# Autodesk Inventor assembly: Assembly2
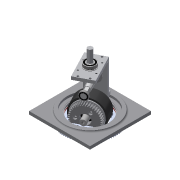
[picture p0: Inventor's stored thumbnail of the model, 180x180]
Saved by Autodesk Inventor 2014 SP1 (Build 180222100, 222)
## iProperties
Created: 2014-04-22
Part Number: Assembly2
Document SubType Name: Assembly
Designer: Rauhul Varma
Author: Rauhul Varma
## Documents named in this file (28)
- C:\Users\Rauhul Varma\Desktop\GRT 2013-2014 Designs\Low CoG Swerve\Assembly2.iam
- C:\Users\Rauhul Varma\Desktop\GRT 2013-2014 Designs\Low CoG Swerve\84T 20 DP Gear.ipt
- C:\Users\Rauhul Varma\Desktop\GRT 2013-2014 Designs\Low CoG Swerve\Module Side Beam.ipt
- C:\Users\Rauhul Varma\Desktop\GRT 2013-2014 Designs\Low CoG Swerve\Wheel.ipt
- C:\Users\Rauhul Varma\Desktop\GRT 2013-2014 Designs\Low CoG Swerve\6901-2RS.ipt
- C:\Users\Rauhul Varma\Desktop\GRT 2013-2014 Designs\Low CoG Swerve\Dead Axle.ipt
- C:\Users\Rauhul Varma\Desktop\GRT 2013-2014 Designs\Low CoG Swerve\FBHCS .25-20 .500 Length.ipt
- C:\Users\Rauhul Varma\Desktop\GRT 2013-2014 Designs\Low CoG Swerve\SHCS LP 8-32 .7500 Long.ipt
- C:\Users\Rauhul Varma\Desktop\GRT 2013-2014 Designs\Low CoG Swerve\SHCS 6-32 .5000 Long.ipt
- C:\Users\Rauhul Varma\Desktop\GRT 2013-2014 Designs\Low CoG Swerve\Dead Axle Spacer.ipt
- C:\Users\Rauhul Varma\Desktop\GRT 2013-2014 Designs\Low CoG Swerve\20T 20 DP Miter Gear.ipt
- C:\Users\Rauhul Varma\Desktop\GRT 2013-2014 Designs\Low CoG Swerve\Needle Roller Assembly.iam
- C:\Users\Rauhul Varma\Desktop\GRT 2013-2014 Designs\Low CoG Swerve\40T 20 DP Spur Gear.ipt
- C:\Users\Rauhul Varma\Desktop\GRT 2013-2014 Designs\Low CoG Swerve\34T 20 DP Spur Gear.ipt
- C:\Users\Rauhul Varma\Desktop\GRT 2013-2014 Designs\Low CoG Swerve\Tread.ipt
- C:\Users\Rauhul Varma\Desktop\GRT 2013-2014 Designs\Low CoG Swerve\689-2RS.ipt
- C:\Users\Rauhul Varma\Desktop\GRT 2013-2014 Designs\Low CoG Swerve\Module Live Axle.ipt
- C:\Users\Rauhul Varma\Desktop\GRT 2013-2014 Designs\Low CoG Swerve\Module Live Axle Thrust Bearing Bushing.ipt
- C:\Users\Rauhul Varma\Desktop\GRT 2013-2014 Designs\Low CoG Swerve\Module Top Plate.ipt
- C:\Users\Rauhul Varma\Desktop\GRT 2013-2014 Designs\Low CoG Swerve\Module Top Cap.ipt
- C:\Users\Rauhul Varma\Desktop\GRT 2013-2014 Designs\Low CoG Swerve\Module Live Axle Gear Spacer.ipt
- C:\Users\Rauhul Varma\Desktop\GRT 2013-2014 Designs\Low CoG Swerve\Module Top Shaft.ipt
- C:\Users\Rauhul Varma\Desktop\GRT 2013-2014 Designs\Low CoG Swerve\Module Top Axle Thrust Bearing Bushing.ipt
- C:\Users\Rauhul Varma\Desktop\GRT 2013-2014 Designs\Low CoG Swerve\6816-2RS.ipt
- C:\Users\Rauhul Varma\Desktop\GRT 2013-2014 Designs\Low CoG Swerve\Swerve Pre Baseplate.ipt
- C:\Users\Rauhul Varma\Desktop\GRT 2013-2014 Designs\Low CoG Swerve\NTA4860 Thrust Bearing.ipt
- C:\Users\Rauhul Varma\Desktop\GRT 2013-2014 Designs\Low CoG Swerve\TRA4860 Thrust Washer.ipt
- C:\Users\Rauhul Varma\Desktop\GRT 2013-2014 Designs\Low CoG Swerve\Bearing Retention Plate.ipt
## Components (44 placed, 27 different names)
1. 84T 20 DP Gear:1 — Mate:1, Mate:2, Mate:3, Mate:4, Mate:5, Mate:6, Mate:17, Mate:35, Mate:36, Mate:37, Mate:38, Mate:39, Mate:40, Mate:41, Mate:42, Mate:110, Mate:111
2. Module Side Beam:1 — Mate:4, Mate:5, Mate:6, Mate:14, Mate:73, Mate:75, Mate:83, Mate:122, Mate:123, Mate:124
3. Module Side Beam:2 — Mate:1, Mate:2, Mate:3, Mate:34, Mate:74, Mate:85, Flush:7, Mate:107, Mate:119, Mate:120, Mate:121
4. Wheel:1 — Mate:14, Mate:17, Mate:18, Mate:19, Mate:20, Mate:21, Mate:62, Mate:69, Mate:71, Mate:72, Mate:125
5. 6901-2RS:1 — Mate:18, Mate:21, Mate:54
6. 6901-2RS:2 — Mate:19, Mate:20, Mate:29, Mate:55
7. Dead Axle:1 — Mate:29, Mate:30, Mate:31, Mate:32, Mate:33, Mate:52, Mate:53
8. FBHCS .25-20 .500 Length:1 — Mate:31, Mate:32, Mate:34
9. FBHCS .25-20 .500 Length:2 — Mate:30, Mate:33
10. SHCS LP 8-32 .7500 Long:1 — Mate:36, Mate:41
11. SHCS LP 8-32 .7500 Long:2 — Mate:37, Mate:40
12. SHCS LP 8-32 .7500 Long:3 — Mate:35, Mate:42
13. SHCS LP 8-32 .7500 Long:4 — Mate:38, Mate:39
14. SHCS 6-32 .5000 Long:1
15. SHCS 6-32 .5000 Long:2
16. SHCS 6-32 .5000 Long:3
17. SHCS 6-32 .5000 Long:4
18. Dead Axle Spacer:1 — Mate:52, Mate:55, Mate:67
19. Dead Axle Spacer:2 — Mate:53, Mate:54
20. 20T 20 DP Miter Gear:1 — Mate:62, Mate:64, Mate:65, Mate:73, Angle:2, Mate:93
21. 20T 20 DP Miter Gear:2 — Mate:64, Mate:65, Mate:81, Mate:82, Mate:99, Mate:100, Mate:102, Mate:106
22. 40T 20 DP Spur Gear:1 — Mate:67, Mate:69, Flush:1, Mate:125
23. 34T 20 DP Spur Gear:1 — Flush:1, Mate:78, Angle:1
24. Tread:1 — Mate:71, Mate:72
25. 689-2RS:1 — Mate:75, Mate:79, Mate:80, Flush:8
26. 689-2RS:2 — Mate:74, Mate:76, Mate:78, Flush:6, Flush:7, Mate:96
27. Needle Roller Assembly:2 [sub-assembly] — Mate:76, Mate:93
28. Module Live Axle:1 — Mate:80, Angle:1, Angle:2, Flush:6, Flush:8, Mate:94, Mate:95
29. Module Live Axle Thrust Bearing Bushing:1 — Mate:79, Mate:94
30. Needle Roller Assembly:3 [sub-assembly] — Mate:81, Mate:82
31. Module Top Plate:1 — Mate:83, Mate:85, Mate:86, Mate:87, Mate:89, Mate:91, Mate:92, Mate:107
32. 6901-2RS:3 — Mate:86, Mate:87
33. Module Top Cap:1 — Mate:88, Mate:89, Mate:90, Mate:91, Mate:92
34. 6901-2RS:4 — Mate:88, Mate:90, Mate:103, Mate:104, Mate:108
35. Module Live Axle Gear Spacer:1 — Mate:95, Mate:96
36. Module Top Shaft:1 — Mate:99, Mate:100, Mate:101, Mate:103, Mate:104
37. Module Top Axle Thrust Bearing Bushing:1 — Mate:101, Mate:102
38. 6816-2RS:1 — Mate:106, Mate:109, Mate:112
39. Swerve Pre Baseplate:1 — Mate:108, Mate:109, Mate:116, Mate:117, Mate:118, Flush:9
40. NTA4860 Thrust Bearing:1 — Mate:112, Mate:113, Mate:114, Mate:115
41. TRA4860 Thrust Washer:1 — Mate:114, Mate:115, Mate:116
42. TRA4860 Thrust Washer:4 — Mate:110, Mate:111, Mate:113
43. Bearing Retention Plate:1 — Mate:122, Mate:123, Mate:124
44. Bearing Retention Plate:2 — Mate:119, Mate:120, Mate:121
## Relationships (92: Mate 85, Flush 5, Angle 2)
- Mate:1: 84T 20 DP Gear:1 ↔ Module Side Beam:2
- Mate:2: 84T 20 DP Gear:1 ↔ Module Side Beam:2
- Mate:3: 84T 20 DP Gear:1 ↔ Module Side Beam:2
- Mate:4: 84T 20 DP Gear:1 ↔ Module Side Beam:1
- Mate:5: 84T 20 DP Gear:1 ↔ Module Side Beam:1
- Mate:6: 84T 20 DP Gear:1 ↔ Module Side Beam:1
- Mate:14: Module Side Beam:1 ↔ Wheel:1
- Mate:17 (1.27 mm): 84T 20 DP Gear:1 ↔ Wheel:1
- Mate:18: Wheel:1 ↔ 6901-2RS:1
- Mate:19: Wheel:1 ↔ 6901-2RS:2
- Mate:20: Wheel:1 ↔ 6901-2RS:2
- Mate:21: Wheel:1 ↔ 6901-2RS:1
- Mate:29: 6901-2RS:2 ↔ Dead Axle:1
- Mate:30: Dead Axle:1 ↔ FBHCS .25-20 .500 Length:2
- Mate:31: Dead Axle:1 ↔ FBHCS .25-20 .500 Length:1
- Mate:32: Dead Axle:1 ↔ FBHCS .25-20 .500 Length:1
- Mate:33: Dead Axle:1 ↔ FBHCS .25-20 .500 Length:2
- Mate:34: Module Side Beam:2 ↔ FBHCS .25-20 .500 Length:1
- Mate:35: 84T 20 DP Gear:1 ↔ SHCS LP 8-32 .7500 Long:3
- Mate:36: 84T 20 DP Gear:1 ↔ SHCS LP 8-32 .7500 Long:1
- Mate:37: 84T 20 DP Gear:1 ↔ SHCS LP 8-32 .7500 Long:2
- Mate:38: 84T 20 DP Gear:1 ↔ SHCS LP 8-32 .7500 Long:4
- Mate:39: 84T 20 DP Gear:1 ↔ SHCS LP 8-32 .7500 Long:4
- Mate:40: 84T 20 DP Gear:1 ↔ SHCS LP 8-32 .7500 Long:2
- Mate:41: 84T 20 DP Gear:1 ↔ SHCS LP 8-32 .7500 Long:1
- Mate:42: 84T 20 DP Gear:1 ↔ SHCS LP 8-32 .7500 Long:3
- Mate:52: Dead Axle:1 ↔ Dead Axle Spacer:1
- Mate:53: Dead Axle:1 ↔ Dead Axle Spacer:2
- Mate:54: 6901-2RS:1 ↔ Dead Axle Spacer:2
- Mate:55: 6901-2RS:2 ↔ Dead Axle Spacer:1
- Mate:62: Wheel:1 ↔ 20T 20 DP Miter Gear:1
- Mate:64: 20T 20 DP Miter Gear:1 ↔ 20T 20 DP Miter Gear:2
- Mate:65: 20T 20 DP Miter Gear:1 ↔ 20T 20 DP Miter Gear:2
- Mate:67: Dead Axle Spacer:1 ↔ 40T 20 DP Spur Gear:1
- Mate:69: Wheel:1 ↔ 40T 20 DP Spur Gear:1
- Flush:1: 40T 20 DP Spur Gear:1 ↔ 34T 20 DP Spur Gear:1
- Mate:71: Wheel:1 ↔ Tread:1
- Mate:72: Wheel:1 ↔ Tread:1
- Mate:73: Module Side Beam:1 ↔ 20T 20 DP Miter Gear:1
- Mate:74: Module Side Beam:2 ↔ 689-2RS:2
- Mate:75: Module Side Beam:1 ↔ 689-2RS:1
- Mate:76: 689-2RS:2 ↔ Needle Roller Assembly:2
- Mate:78: 34T 20 DP Spur Gear:1 ↔ 689-2RS:2
- Mate:79: 689-2RS:1 ↔ Module Live Axle Thrust Bearing Bushing:1
- Mate:80: 689-2RS:1 ↔ Module Live Axle:1
- Angle:1 (0 deg): 34T 20 DP Spur Gear:1 ↔ Module Live Axle:1
- Angle:2 (0 deg): 20T 20 DP Miter Gear:1 ↔ Module Live Axle:1
- Flush:6: 689-2RS:2 ↔ Module Live Axle:1
- Mate:81: 20T 20 DP Miter Gear:2 ↔ Needle Roller Assembly:3
- Mate:82: 20T 20 DP Miter Gear:2 ↔ Needle Roller Assembly:3
- Mate:83: Module Side Beam:1 ↔ Module Top Plate:1
- Mate:85: Module Side Beam:2 ↔ Module Top Plate:1
- Mate:86: Module Top Plate:1 ↔ 6901-2RS:3
- Mate:87: Module Top Plate:1 ↔ 6901-2RS:3
- Mate:88: Module Top Cap:1 ↔ 6901-2RS:4
- Mate:89: Module Top Plate:1 ↔ Module Top Cap:1
- Mate:90: Module Top Cap:1 ↔ 6901-2RS:4
- Mate:91: Module Top Plate:1 ↔ Module Top Cap:1
- Mate:92: Module Top Plate:1 ↔ Module Top Cap:1
- Flush:7: Module Side Beam:2 ↔ 689-2RS:2
- Mate:93: 20T 20 DP Miter Gear:1 ↔ Needle Roller Assembly:2
- Flush:8: 689-2RS:1 ↔ Module Live Axle:1
- Mate:94: Module Live Axle:1 ↔ Module Live Axle Thrust Bearing Bushing:1
- Mate:95: Module Live Axle:1 ↔ Module Live Axle Gear Spacer:1
- Mate:96: 689-2RS:2 ↔ Module Live Axle Gear Spacer:1
- Mate:99: 20T 20 DP Miter Gear:2 ↔ Module Top Shaft:1
- Mate:100: 20T 20 DP Miter Gear:2 ↔ Module Top Shaft:1
- Mate:101: Module Top Shaft:1 ↔ Module Top Axle Thrust Bearing Bushing:1
- Mate:102: 20T 20 DP Miter Gear:2 ↔ Module Top Axle Thrust Bearing Bushing:1
- Mate:103: 6901-2RS:4 ↔ Module Top Shaft:1
- Mate:104: 6901-2RS:4 ↔ Module Top Shaft:1
- Mate:106: 20T 20 DP Miter Gear:2 ↔ 6816-2RS:1
- Mate:107: Module Side Beam:2 ↔ Module Top Plate:1
- Mate:108: 6901-2RS:4 ↔ Swerve Pre Baseplate:1
- Mate:109: 6816-2RS:1 ↔ Swerve Pre Baseplate:1
- Mate:110: 84T 20 DP Gear:1 ↔ TRA4860 Thrust Washer:4
- Mate:111: 84T 20 DP Gear:1 ↔ TRA4860 Thrust Washer:4
- Mate:112: 6816-2RS:1 ↔ NTA4860 Thrust Bearing:1
- Mate:113: NTA4860 Thrust Bearing:1 ↔ TRA4860 Thrust Washer:4
- Mate:114: NTA4860 Thrust Bearing:1 ↔ TRA4860 Thrust Washer:1
- Mate:115: NTA4860 Thrust Bearing:1 ↔ TRA4860 Thrust Washer:1
- Mate:116: Swerve Pre Baseplate:1 ↔ TRA4860 Thrust Washer:1
- Mate:117: Swerve Pre Baseplate:1
- Mate:118: Swerve Pre Baseplate:1
- Flush:9: Swerve Pre Baseplate:1
- Mate:119: Module Side Beam:2 ↔ Bearing Retention Plate:2
- Mate:120: Module Side Beam:2 ↔ Bearing Retention Plate:2
- Mate:121: Module Side Beam:2 ↔ Bearing Retention Plate:2
- Mate:122: Module Side Beam:1 ↔ Bearing Retention Plate:1
- Mate:123: Module Side Beam:1 ↔ Bearing Retention Plate:1
- Mate:124: Module Side Beam:1 ↔ Bearing Retention Plate:1
- Mate:125: Wheel:1 ↔ 40T 20 DP Spur Gear:1
